# Autodesk Inventor assembly: Engine skin glued
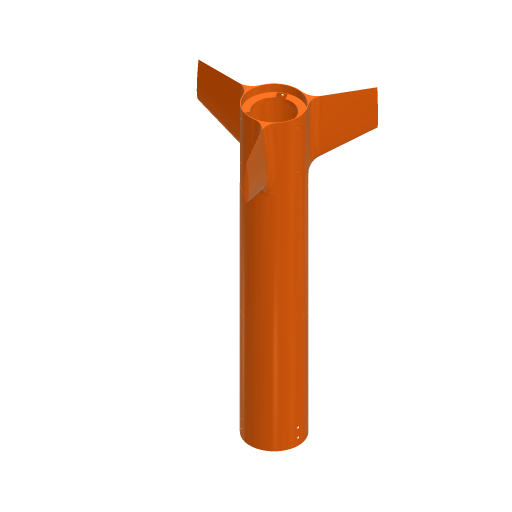
[picture p0: Inventor's stored thumbnail of the model, 512x512]
Saved by Autodesk Inventor 2024 (Build 280153000, 153)
## iProperties
Created: 2024-01-03
Part Number: Engine skin glued
Document SubType Name: Assembly
Designer: Jamie
Mass: 154.6 g
Surface Area: 2298.95 cm^2
Volume: 162.395 cm^3
Density: 0.952 g/cm^3
Author: Jamie
## Documents named in this file (4)
- C:\Users\Jamie\Documents\Uni\DARE\Scrambler-2-CAD\Autodesk\Engine skin glued.iam
- C:\Users\Jamie\Documents\Uni\DARE\Scrambler-2-CAD\Autodesk\Engine lower skin.ipt
- C:\Users\Jamie\Documents\Uni\DARE\Scrambler-2-CAD\Autodesk\Engine upper skin.ipt
- C:\Users\Jamie\Documents\Uni\DARE\Scrambler-2-CAD\Autodesk\Fins.ipt
## Components (3 placed, 3 different names)
1. Engine lower skin:1 — Mate:1, Mate:2, Mate:3, Mate:4
2. Engine upper skin:1 — Mate:3, Mate:4, Angle:1
3. Fins:1 — Mate:1, Mate:2, Angle:1
## Relationships (5: Mate 4, Angle 1)
- Mate:1: Engine lower skin:1 ↔ Fins:1
- Mate:2: Engine lower skin:1 ↔ Fins:1
- Mate:3: Engine lower skin:1 ↔ Engine upper skin:1
- Mate:4: Engine lower skin:1 ↔ Engine upper skin:1
- Angle:1 (60 deg): Engine upper skin:1 ↔ Fins:1
